# Autodesk Inventor assembly: Simulation_module_2
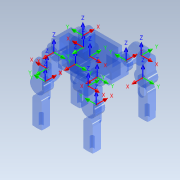
[picture p0: Inventor's stored thumbnail of the model, 180x180]
Saved by Autodesk Inventor 2020 (Build 240168000, 168)
## iProperties
Created: 2021-01-12
Part Number: Simulation_module_2
Document SubType Name: Assembly
Designer: DELL
Author: DELL
## Documents named in this file (6)
- F:\SoftRobot2.0\FlexipodHardware2.0\FlexipodHardware\Flexipod2.0\Cadquery_module\Simulation_module_2.iam
- F:\SoftRobot2.0\FlexipodHardware2.0\FlexipodHardware\Flexipod2.0\Cadquery_module\body_inventor.ipt
- F:\SoftRobot2.0\FlexipodHardware2.0\FlexipodHardware\Flexipod2.0\Cadquery_module\hip_inventor.ipt
- F:\SoftRobot2.0\FlexipodHardware2.0\FlexipodHardware\Flexipod2.0\Cadquery_module\thigh_inventor.ipt
- F:\SoftRobot2.0\FlexipodHardware2.0\FlexipodHardware\Flexipod2.0\Cadquery_module\shank_inventor.ipt
- F:\SoftRobot2.0\FlexipodHardware2.0\FlexipodHardware\Flexipod2.0\Cadquery_module\hip_inventor_back.ipt
## Components (13 placed, 5 different names)
1. body_inventor:1 — Mate:1, Mate:2, Flush:1, Flush:2, Flush:3, Angle:1, Angle:2, Angle:3, Mate:7, Mate:8, Angle:4, Angle:5, Mate:13, Mate:14, Angle:7, Mate:15, Mate:16, Angle:8
2. hip_inventor:1 — Mate:1, Mate:2, Angle:1, Mate:3, Mate:4
3. hip_inventor:2 — Mate:7, Mate:8, Angle:4, Mate:9, Mate:10
4. thigh_inventor:1 — Mate:3, Mate:4, Angle:2, Mate:5, Mate:6, Flush:4
5. thigh_inventor:2 — Mate:9, Mate:10, Angle:5, Mate:11, Mate:12, Angle:6
6. shank_inventor:1 — Mate:11, Mate:12, Angle:6
7. shank_inventor:2 — Mate:5, Mate:6, Angle:3, Flush:5
8. hip_inventor_back:1 — Mate:13, Mate:14, Angle:7, Mate:17, Mate:18, Angle:9, Flush:7
9. hip_inventor_back:2 — Mate:15, Mate:16, Angle:8, Mate:19, Mate:20, Angle:10
10. thigh_inventor:3 — Mate:17, Mate:18, Angle:9, Mate:23, Mate:24, Angle:12
11. thigh_inventor:4 — Mate:19, Mate:20, Angle:10, Mate:21, Mate:22, Angle:11
12. shank_inventor:3 — Mate:21, Mate:22, Angle:11
13. shank_inventor:4 — Mate:23, Mate:24, Angle:12, Flush:6
## Relationships (43: Mate 24, Angle 12, Flush 7)
- Mate:1: body_inventor:1 ↔ hip_inventor:1
- Mate:2: body_inventor:1 ↔ hip_inventor:1
- Flush:1: body_inventor:1
- Flush:2: body_inventor:1
- Flush:3: body_inventor:1
- Angle:1 (0 deg): body_inventor:1 ↔ hip_inventor:1
- Mate:3 (-10.5 mm): hip_inventor:1 ↔ thigh_inventor:1
- Mate:4: hip_inventor:1 ↔ thigh_inventor:1
- Angle:2 (0 deg): body_inventor:1 ↔ thigh_inventor:1
- Mate:5 (-9 mm): thigh_inventor:1 ↔ shank_inventor:2
- Mate:6: thigh_inventor:1 ↔ shank_inventor:2
- Angle:3 (0 deg): body_inventor:1 ↔ shank_inventor:2
- Mate:7: body_inventor:1 ↔ hip_inventor:2
- Mate:8: body_inventor:1 ↔ hip_inventor:2
- Angle:4 (0 deg): body_inventor:1 ↔ hip_inventor:2
- Mate:9 (-10.5 mm): hip_inventor:2 ↔ thigh_inventor:2
- Mate:10: hip_inventor:2 ↔ thigh_inventor:2
- Angle:5 (0 deg): body_inventor:1 ↔ thigh_inventor:2
- Mate:11 (-9 mm): thigh_inventor:2 ↔ shank_inventor:1
- Mate:12: thigh_inventor:2 ↔ shank_inventor:1
- Angle:6 (0 deg): thigh_inventor:2 ↔ shank_inventor:1
- Mate:13: body_inventor:1 ↔ hip_inventor_back:1
- Mate:14: body_inventor:1 ↔ hip_inventor_back:1
- Angle:7 (0 deg): body_inventor:1 ↔ hip_inventor_back:1
- Mate:15: body_inventor:1 ↔ hip_inventor_back:2
- Mate:16: body_inventor:1 ↔ hip_inventor_back:2
- Angle:8 (0 deg): body_inventor:1 ↔ hip_inventor_back:2
- Mate:17 (-9 mm): hip_inventor_back:1 ↔ thigh_inventor:3
- Mate:18: hip_inventor_back:1 ↔ thigh_inventor:3
- Angle:9 (0 deg): hip_inventor_back:1 ↔ thigh_inventor:3
- Mate:19 (-9 mm): hip_inventor_back:2 ↔ thigh_inventor:4
- Mate:20: hip_inventor_back:2 ↔ thigh_inventor:4
- Angle:10 (0 deg): hip_inventor_back:2 ↔ thigh_inventor:4
- Mate:21 (-9 mm): thigh_inventor:4 ↔ shank_inventor:3
- Mate:22: thigh_inventor:4 ↔ shank_inventor:3
- Angle:11 (0 deg): thigh_inventor:4 ↔ shank_inventor:3
- Mate:23 (-9 mm): thigh_inventor:3 ↔ shank_inventor:4
- Mate:24: thigh_inventor:3 ↔ shank_inventor:4
- Angle:12 (0 deg): thigh_inventor:3 ↔ shank_inventor:4
- Flush:4: thigh_inventor:1
- Flush:5: shank_inventor:2
- Flush:6: shank_inventor:4
- Flush:7: hip_inventor_back:1
